# Autodesk Inventor assembly: Ensamble herramienta
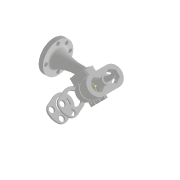
[picture p0: Inventor's stored thumbnail of the model, 180x180]
Saved by Autodesk Inventor 2022 (Build 260153000, 153)
## iProperties
Created: 2022-11-24
Part Number: Ensamble herramienta
Document SubType Name: Assembly
Designer: ADMIN
Author: ADMIN
## Documents named in this file (7)
- G:\Unidades compartidas\Amiguitos por siempre\Robotica\Proyecto final\Herramienta\Ensamble herramienta.iam
- G:\Unidades compartidas\Amiguitos por siempre\Robotica\Proyecto final\Herramienta\Porta herramientas p1.ipt
- G:\Unidades compartidas\Amiguitos por siempre\Robotica\Proyecto final\Herramienta\Porta herramientas p2.ipt
- G:\Unidades compartidas\Amiguitos por siempre\Robotica\Proyecto final\Herramienta\Sujeción mangueras.ipt
- G:\Unidades compartidas\Amiguitos por siempre\Robotica\Proyecto final\Herramienta\Sujeción venturi a ventosa.ipt
- G:\Unidades compartidas\Amiguitos por siempre\Robotica\Proyecto final\Herramienta\Acople Venturi.ipt
- G:\Unidades compartidas\Amiguitos por siempre\Robotica\Proyecto final\Herramienta\Punta calibración 2.ipt
## Components (9 placed, 6 different names)
1. Porta herramientas p1:1 — Mate:2, Mate:3
2. Porta herramientas p2:1 — Mate:2, Mate:3, Mate:4, Angle:1, Mate:7, Angle:3
3. Sujeción mangueras:1 — Mate:8, Mate:9, Mate:10
4. Sujeción venturi a ventosa:1 — Angle:2, Mate:11, Mate:12, Angle:3
5. Acople Venturi:1 — Mate:4, Mate:5, Mate:6, Flush:2, Mate:8, Angle:2, Mate:11
6. Acople Venturi:2 — Mate:5, Flush:1, Flush:2, Angle:1, Mate:7
7. Acople Venturi:3 — Mate:6, Flush:1
8. Sujeción mangueras:2 — Mate:9, Mate:10
9. Punta calibración 2:1 — Mate:12
## Relationships (16: Mate 11, Angle 3, Flush 2)
- Mate:2: Porta herramientas p1:1 ↔ Porta herramientas p2:1
- Mate:3: Porta herramientas p1:1 ↔ Porta herramientas p2:1
- Mate:4: Porta herramientas p2:1 ↔ Acople Venturi:1
- Mate:5: Acople Venturi:1 ↔ Acople Venturi:2
- Mate:6: Acople Venturi:1 ↔ Acople Venturi:3
- Flush:1: Acople Venturi:2 ↔ Acople Venturi:3
- Flush:2: Acople Venturi:1 ↔ Acople Venturi:2
- Angle:1 (0 deg): Porta herramientas p2:1 ↔ Acople Venturi:2
- Mate:7 (0.3 mm): Porta herramientas p2:1 ↔ Acople Venturi:2
- Mate:8: Sujeción mangueras:1 ↔ Acople Venturi:1
- Mate:9: Sujeción mangueras:1 ↔ Sujeción mangueras:2
- Mate:10: Sujeción mangueras:1 ↔ Sujeción mangueras:2
- Angle:2 (0 deg): Sujeción venturi a ventosa:1 ↔ Acople Venturi:1
- Mate:11: Sujeción venturi a ventosa:1 ↔ Acople Venturi:1
- Mate:12: Sujeción venturi a ventosa:1 ↔ Punta calibración 2:1
- Angle:3 (0 deg): Porta herramientas p2:1 ↔ Sujeción venturi a ventosa:1
